# Autodesk Inventor assembly: mixer
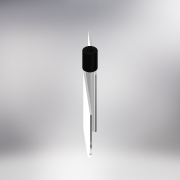
[picture p0: Inventor's stored thumbnail of the model, 180x180]
Saved by Autodesk Inventor 2020 (Build 240168000, 168)
## iProperties
Created: 2020-06-18
Part Number: mixer
Document SubType Name: Assembly
Designer: pc-konvi
Author: pc-konvi
## Documents named in this file (4)
- C:\Users\pc-konvi\Documents\Lobola\open_source_scrabble\lobola - rapid prototype\mixer.iam
- C:\Users\pc-konvi\Documents\Lobola\open_source_scrabble\lobola - rapid prototype\blade.ipt
- C:\Users\pc-konvi\Documents\Lobola\open_source_scrabble\lobola - rapid prototype\blade_rod.ipt
- C:\Users\pc-konvi\Documents\Lobola\open_source_scrabble\lobola - rapid prototype\mixer_coupler.ipt
## Components (4 placed, 3 different names)
1. blade_rod:1 — Mate:10, Mate:11, Flush:12, Flush:13, Mate:19
2. mixer_coupler:1 — Mate:10, Mate:11, Flush:15
3. blade:2 — Mate:16, Flush:12, Flush:13, Flush:14, Mate:17, Mate:18
4. blade:3 — Flush:14, Mate:17, Mate:18
## Relationships (10: Mate 6, Flush 4)
- Mate:10: blade_rod:1 ↔ mixer_coupler:1
- Mate:11: blade_rod:1 ↔ mixer_coupler:1
- Mate:16 (4 mm): blade:2
- Flush:12: blade_rod:1 ↔ blade:2
- Flush:13 (-4 mm): blade_rod:1 ↔ blade:2
- Flush:14: blade:2 ↔ blade:3
- Mate:17 (8 mm): blade:2 ↔ blade:3
- Mate:18 (-8 mm): blade:2 ↔ blade:3
- Mate:19: blade_rod:1
- Flush:15: mixer_coupler:1
